# Autodesk Inventor assembly: Assembly1
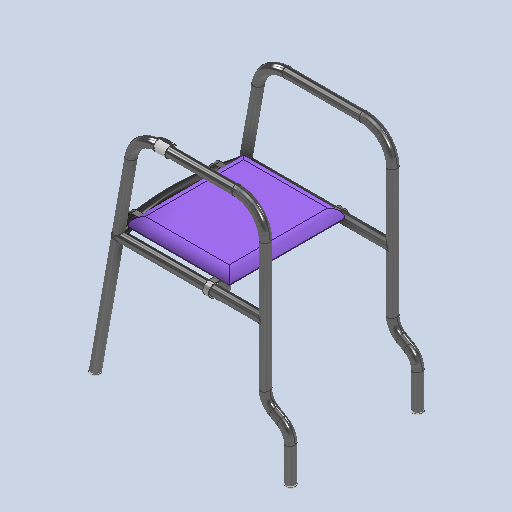
[picture p0: Inventor's stored thumbnail of the model, 512x512]
Saved by Autodesk Inventor 2025.2 (Build 292293000, 293)
## iProperties
Created: 2024-05-29
Part Number: Assembly1
Document SubType Name: Assembly
Designer: mirun
Author: mirun
## Documents named in this file (7)
- C:\Users\mirewn\OneDrive - Universitatea Politehnica Bucuresti\AA- Projects\Scaun estetica\Assembly1.iam
- C:\Users\mirewn\OneDrive - Universitatea Politehnica Bucuresti\AA- Projects\Scaun estetica\frame.ipt
- C:\Users\mirewn\OneDrive - Universitatea Politehnica Bucuresti\AA- Projects\Scaun estetica\leg_ends.ipt
- C:\Users\mirewn\OneDrive - Universitatea Politehnica Bucuresti\AA- Projects\Scaun estetica\cushions.ipt
- C:\Users\mirewn\OneDrive - Universitatea Politehnica Bucuresti\AA- Projects\Scaun estetica\seat.ipt
- C:\Users\mirewn\OneDrive - Universitatea Politehnica Bucuresti\AA- Projects\Scaun estetica\monitor.ipt
- C:\Users\mirewn\OneDrive - Universitatea Politehnica Bucuresti\AA- Projects\Scaun estetica\screen.ipt
## Components (9 placed, 6 different names)
1. frame:1 — Mate:1, Mate:2, Mate:3, Mate:4, Mate:5, Mate:13, Mate:14, Mate:15, Mate:16
2. leg_ends:1 — Mate:1, Mate:2, Flush:1
3. leg_ends:2 — Mate:5
4. leg_ends:3 — Mate:4
5. leg_ends:4 — Mate:3
6. cushions:1 — Mate:6, Mate:8, Mate:9
7. seat:1 — Mate:6, Mate:8, Mate:9, Mate:15, Mate:16
8. monitor:1 — Mate:11, Mate:12, Mate:13, Mate:14
9. screen:1 — Mate:11, Mate:12
## Relationships (15: Mate 14, Flush 1)
- Mate:1: frame:1 ↔ leg_ends:1
- Mate:2: frame:1 ↔ leg_ends:1
- Mate:3: frame:1 ↔ leg_ends:4
- Mate:4: frame:1 ↔ leg_ends:3
- Mate:5: frame:1 ↔ leg_ends:2
- Mate:6: cushions:1 ↔ seat:1
- Mate:8: cushions:1 ↔ seat:1
- Flush:1 (466 mm): leg_ends:1
- Mate:9: cushions:1 ↔ seat:1
- Mate:11: monitor:1 ↔ screen:1
- Mate:12: monitor:1 ↔ screen:1
- Mate:13: frame:1 ↔ monitor:1
- Mate:14: frame:1 ↔ monitor:1
- Mate:15: frame:1 ↔ seat:1
- Mate:16: frame:1 ↔ seat:1
